# Autodesk Inventor assembly: Basurero
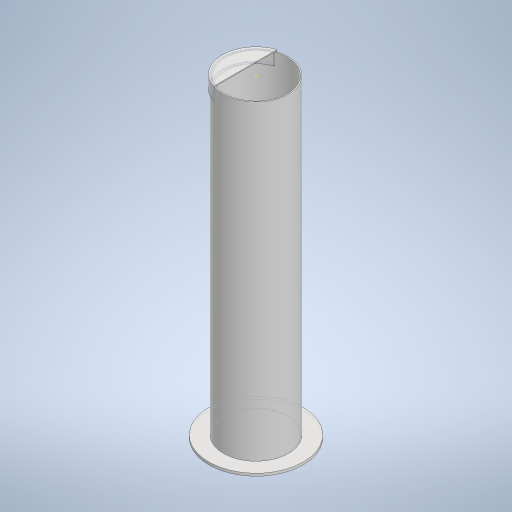
[picture p0: Inventor's stored thumbnail of the model, 512x512]
Saved by Autodesk Inventor 2024 (Build 280153000, 153)
## iProperties
Created: 2024-05-21
Part Number: Basurero
Document SubType Name: Assembly
Designer: psepu
Author: psepu
## Documents named in this file (3)
- C:\Users\psepu\OneDrive\Documentos\U. Lorraine Francia\Basurero.iam
- C:\Users\psepu\OneDrive\Documentos\U. Lorraine Francia\Cuerpo.ipt
- C:\Users\psepu\OneDrive\Documentos\U. Lorraine Francia\Tapa2.ipt
## Components (2 placed, 2 different names)
1. Cuerpo:1 — De rotación:1
2. Tapa2:1 — De rotación:1
## Relationships (1: RevoluteJoint 1)
- De rotación:1 [RevoluteJoint]: Cuerpo:1 ↔ Tapa2:1
